# Autodesk Inventor assembly: Prensa_Hidraulica
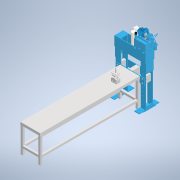
[picture p0: Inventor's stored thumbnail of the model, 180x180]
Saved by Autodesk Inventor 2021 (Build 250183000, 183)
## iProperties
Created: 2020-01-15
Part Number: Prensa_Hidraulica
Document SubType Name: Assembly
Designer: Nelson
Sending System: SolidWorks 2020
Last Author: Micro
Last Saved: 2020-01-16
Author: Nelson
## Documents named in this file (10)
- D:\Nelson\Documentos\Inventor\PrensaHidraulica_Automatizada\Prensa_Hidraulica.iam
- Prensa_Hidraulica.iam
- D:\Nelson\Documentos\Inventor\PrensaHidraulica_Automatizada\Estructura.iam
- D:\Nelson\Documentos\Inventor\PrensaHidraulica_Automatizada\Cilindro neumatico.ipt
- D:\Nelson\Documentos\Inventor\PrensaHidraulica_Automatizada\Bomba Hidraulica.ipt
- D:\Nelson\Documentos\Inventor\PrensaHidraulica_Automatizada\Soporte barras.ipt
- D:\Nelson\Documentos\Inventor\PrensaHidraulica_Automatizada\Ensamble Mecanismo cilindro.iam
- D:\Nelson\Documentos\Inventor\PrensaHidraulica_Automatizada\Soporte mesa.ipt
- D:\Nelson\Documentos\Inventor\PrensaHidraulica_Automatizada\PH 013.ipt
- D:\Nelson\Documentos\Inventor\PrensaHidraulica_Automatizada\Mesa.iam
## Components (12 placed, 8 different names)
1. Cilindro neumatico:1 — Mate:2, Mate:3
2. Bomba Hidraulica:1 — Mate:1, Flush:1, Flush:2
3. Soporte barras:1 — Mate:4, Mate:19
4. Soporte barras:2 — Mate:5, Mate:20
5. Soporte mesa:1 — Mate:29, Mate:30, Mate:31
6. PH 013:3 — Mate:40, Mate:42
7. PH 013:4 — Mate:41, Mate:43
8. PH 013:5 — Mate:34, Mate:35
9. PH 013:6 — Mate:32, Mate:33
10. Ensamble mecanismo cilindro:1 [sub-assembly]
11. Mesa:1 [sub-assembly] — Flush:3, Mate:44, Mate:45
12. Estructura:1 [sub-assembly] — Mate:1, Flush:1, Flush:2, Mate:2, Mate:3, Mate:4, Mate:5, Mate:19, Mate:20, Mate:29, Mate:30, Mate:31, Mate:32, Mate:33, Mate:34, Mate:35, Mate:40, Mate:41, Mate:42, Mate:43, Flush:3, Mate:44, Mate:45
## Relationships (23: Mate 20, Flush 3)
- Mate:1: Bomba Hidraulica:1 ↔ Estructura:1
- Flush:1: Bomba Hidraulica:1 ↔ Estructura:1
- Flush:2: Bomba Hidraulica:1 ↔ Estructura:1
- Mate:2: Cilindro neumatico:1 ↔ Estructura:1
- Mate:3: Cilindro neumatico:1 ↔ Estructura:1
- Mate:4: Soporte barras:1 ↔ Estructura:1
- Mate:5: Soporte barras:2 ↔ Estructura:1
- Mate:19: Soporte barras:1 ↔ Estructura:1
- Mate:20: Soporte barras:2 ↔ Estructura:1
- Mate:29: Soporte mesa:1 ↔ Estructura:1
- Mate:30: Soporte mesa:1 ↔ Estructura:1
- Mate:31: Soporte mesa:1 ↔ Estructura:1
- Mate:32: PH 013:6 ↔ Estructura:1
- Mate:33: PH 013:6 ↔ Estructura:1
- Mate:34: PH 013:5 ↔ Estructura:1
- Mate:35: PH 013:5 ↔ Estructura:1
- Mate:40: PH 013:3 ↔ Estructura:1
- Mate:41: PH 013:4 ↔ Estructura:1
- Mate:42: PH 013:3 ↔ Estructura:1
- Mate:43: PH 013:4 ↔ Estructura:1
- Flush:3: Mesa:1 ↔ Estructura:1
- Mate:44: Mesa:1 ↔ Estructura:1
- Mate:45: Mesa:1 ↔ Estructura:1
